# Autodesk Inventor assembly: Start of Robot Base
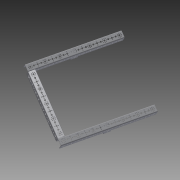
[picture p0: Inventor's stored thumbnail of the model, 180x180]
Saved by Autodesk Inventor 2015 (Build 190159000, 159)
## iProperties
Created: 2015-09-26
Part Number: Start of Robot Base
Document SubType Name: Assembly
Designer: damedin
Author: damedin
## Documents named in this file (3)
- U:\Start of Robot Base.iam
- C:\Users\damedin\Documents\COTS Parts\Tetrix\Tetrix channel 288mm.ipt
- C:\Users\damedin\Documents\COTS Parts\Tetrix\Tetrix Channel 416mm.ipt
## Components (3 placed, 2 different names)
1. Tetrix channel 288mm:1 — Mate:1, Flush:1, Mate:2, Mate:3, Flush:2, Mate:4
2. Tetrix Channel 416mm:1 — Mate:3, Flush:2, Mate:4
3. Tetrix Channel 416mm:2 — Mate:1, Flush:1, Mate:2
## Relationships (6: Mate 4, Flush 2)
- Mate:1: Tetrix channel 288mm:1 ↔ Tetrix Channel 416mm:2
- Flush:1: Tetrix channel 288mm:1 ↔ Tetrix Channel 416mm:2
- Mate:2: Tetrix channel 288mm:1 ↔ Tetrix Channel 416mm:2
- Mate:3: Tetrix channel 288mm:1 ↔ Tetrix Channel 416mm:1
- Flush:2: Tetrix channel 288mm:1 ↔ Tetrix Channel 416mm:1
- Mate:4: Tetrix channel 288mm:1 ↔ Tetrix Channel 416mm:1
